# Autodesk Inventor assembly: RobotWithCatapult
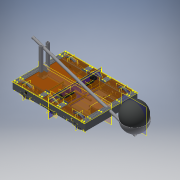
[picture p0: Inventor's stored thumbnail of the model, 180x180]
Saved by Autodesk Inventor 2016 SP1 (Build 200210100, 210)
## iProperties
Created: 2016-01-19
Part Number: RobotWithCatapult
Document SubType Name: Assembly
Designer: steele
Author: steele
## Documents named in this file (11)
- C:\snobotics\CAD-Development\robSteele\SnoBotics2016\2ndCutAtCatapultRobot\RobotWithCatapult.iam
- C:\snobotics\CAD-Development\robSteele\SnoBotics2016\AM 14 U 3 Long\am14u3_long.iam
- C:\snobotics\CAD-Development\robSteele\SnoBotics2016\2ndCutAtCatapultRobot\frontPlate.ipt
- C:\snobotics\CAD-Development\robSteele\SnoBotics2016\2ndCutAtCatapultRobot\catapultArmSupportStructure.ipt
- C:\snobotics\CAD-Development\robSteele\SnoBotics2016\FirstCutCatapult\roundCatapultArm.ipt
- C:\snobotics\CAD-MfgResources\McMaster-Carr\Air Cylinder\Universal Mount\Single Acting Spring Return\3_4 bore 6 stroke\6498K045.ipt
- C:\snobotics\CAD-Development\robSteele\SnoBotics2016\FirstCutCatapult\cArmPully.ipt
- C:\snobotics\CAD-Development\robSteele\SnoBotics2016\FirstCutCatapult\CatapultAxel.ipt
- C:\snobotics\CAD-Development\robSteele\SnoBotics2016\2ndCutAtCatapultRobot\6498K330.ipt
- C:\snobotics\CAD-Development\robSteele\SnoBotics2016\2ndCutAtCatapultRobot\GE-16180_1.ipt
- C:\snobotics\CAD-Development\robSteele\SnoBotics2016\2ndCutAtCatapultRobot\roundSaladBowl.ipt
## Components (11 placed, 10 different names)
1. am14u3_long:1 [sub-assembly] — Mate:2, Mate:3, Mate:4, Mate:6
2. frontPlate:1 — Mate:2, Mate:3, Mate:4, Mate:5, Flush:1, Mate:7, Flush:9, Flush:10, Mate:8
3. catapultArmSupportStructure:1 — Mate:5, Mate:6, Flush:1, Rotational:1, Insert:1, Insert:2
4. roundCatapultArm:1 — Rotational:1
5. 6498K045:1 — Insert:4
6. cArmPully:1 — Insert:3
7. CatapultAxel:1 — Insert:1, Insert:3
8. CatapultAxel:2 — Insert:2
9. 6498K330:1 — Mate:7, Flush:9, Flush:10, Insert:4
10. GE-16180_1:1 — Mate:8
11. roundSaladBowl:1
## Relationships (15: Mate 7, Insert 4, Flush 3, RevoluteJoint 1)
- Mate:2: am14u3_long:1 ↔ frontPlate:1
- Mate:3: am14u3_long:1 ↔ frontPlate:1
- Mate:4: am14u3_long:1 ↔ frontPlate:1
- Mate:5: frontPlate:1 ↔ catapultArmSupportStructure:1
- Mate:6: am14u3_long:1 ↔ catapultArmSupportStructure:1
- Flush:1 (-25.4 mm): frontPlate:1 ↔ catapultArmSupportStructure:1
- Rotational:1 [RevoluteJoint]: catapultArmSupportStructure:1 ↔ roundCatapultArm:1
- Insert:1: catapultArmSupportStructure:1 ↔ CatapultAxel:1
- Insert:2: catapultArmSupportStructure:1 ↔ CatapultAxel:2
- Insert:3 (-12.7 mm): cArmPully:1 ↔ CatapultAxel:1
- Mate:7: frontPlate:1 ↔ 6498K330:1
- Flush:9: frontPlate:1 ↔ 6498K330:1
- Flush:10 (-25.4 mm): frontPlate:1 ↔ 6498K330:1
- Insert:4: 6498K045:1 ↔ 6498K330:1
- Mate:8: frontPlate:1 ↔ GE-16180_1:1
